# Autodesk Inventor assembly: TinyTurner
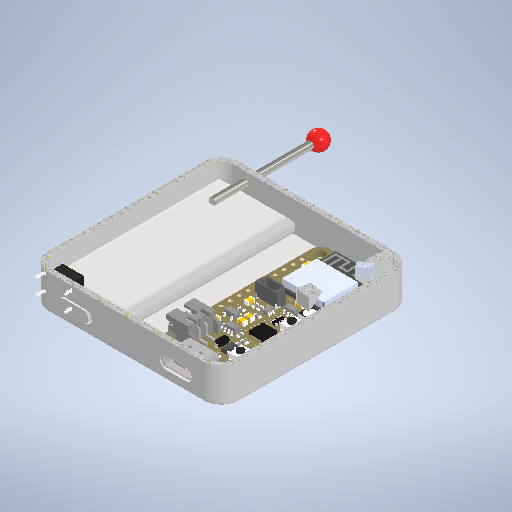
[picture p0: Inventor's stored thumbnail of the model, 512x512]
Saved by Autodesk Inventor 2026 (Build 300175050, 175E)
## iProperties
Created: 2025-07-10
Part Number: TinyTurner
Document SubType Name: Assembly
Designer: Jochen Alt
Author: Jochen Alt
## Documents named in this file (9)
- D:\Projects\TinyTurner\CAD\TinyTurner.iam
- D:\Projects\TinyTurner\CAD\Box.ipt
- D:\Projects\TinyTurner\CAD\Antenna.ipt
- D:\Projects\TinyTurner\CAD\Grid.ipt
- D:\Projects\TinyTurner\CAD\External Components\led-2mm\Led_2mm\Led_2mm\Led_2mm.ipt
- D:\Projects\TinyTurner\CAD\Button Cap.ipt
- D:\Projects\TinyTurner\CAD\External Components\5400 ESP32 Feather V2\5400 ESP32 Feather V2.iam
- D:\Projects\TinyTurner\CAD\External Components\button-6x6\button 6x6\button 6x6\button 6x6.ipt
- D:\Projects\TinyTurner\CAD\3,.7V 500mAh.ipt
## Components (8 placed, 8 different names)
1. Box:1 — Mate:1, Mate:2, Mate:3, Angle:1, Mate:7, Mate:11, Mate:13, Mate:14, Mate:15, Mate:16, Angle:2, Angle:3, Angle:4, Mate:20, Mate:21
2. Antenna:1 — Mate:1, Mate:17
3. Grid:1 — Mate:2, Mate:3
4. Led_2mm:1 — Mate:11, Mate:16
5. Button Cap:1 — Angle:1, Mate:7
6. 5400 ESP32 Feather V2:1 [sub-assembly] — Mate:13, Mate:14, Mate:15
7. button 6x6:1 — Angle:2, Mate:17, Angle:3
8. 3,.7V 500mAh:1 — Angle:4, Mate:20, Mate:21
## Relationships (16: Mate 12, Angle 4)
- Mate:1: Box:1 ↔ Antenna:1
- Mate:2: Box:1 ↔ Grid:1
- Mate:3: Box:1 ↔ Grid:1
- Angle:1 (0 deg): Box:1 ↔ Button Cap:1
- Mate:7: Box:1 ↔ Button Cap:1
- Mate:11: Box:1 ↔ Led_2mm:1
- Mate:13: Box:1 ↔ 5400 ESP32 Feather V2:1
- Mate:14: Box:1 ↔ 5400 ESP32 Feather V2:1
- Mate:15: Box:1 ↔ 5400 ESP32 Feather V2:1
- Mate:16: Box:1 ↔ Led_2mm:1
- Angle:2 (180 deg): Box:1 ↔ button 6x6:1
- Mate:17: Antenna:1 ↔ button 6x6:1
- Angle:3 (0 deg): Box:1 ↔ button 6x6:1
- Angle:4 (0 deg): Box:1 ↔ 3,.7V 500mAh:1
- Mate:20: Box:1 ↔ 3,.7V 500mAh:1
- Mate:21: Box:1 ↔ 3,.7V 500mAh:1
